# Autodesk Inventor assembly: body_8d_wid_1
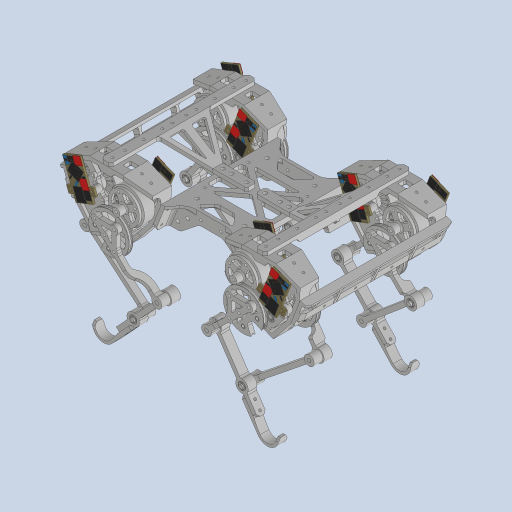
[picture p0: Inventor's stored thumbnail of the model, 512x512]
Saved by Autodesk Inventor 2023 (Build 270158000, 158)
## iProperties
Created: 2021-03-13
Part Number: body_8d_wid_1
Document SubType Name: Assembly
Designer: Shuang Peng
Author: Shuang Peng
## Documents named in this file (6)
- D:\projects-3\biped_tiny\hardware\body_8d_wid_1.iam
- D:\projects-3\biped_tiny\hardware\leg_2d_1.iam
- D:\projects-3\biped_tiny\hardware\leg_1_2d_MIR.iam
- D:\projects-3\biped_tiny\hardware\body_linker_1_wid_8d.ipt
- D:\projects-3\biped_tiny\hardware\body_linker_2_8d_wid.ipt
- D:\projects-3\biped_tiny\hardware\ex_shell_2_wid.ipt
## Components (9 placed, 5 different names)
1. leg_2d_1:1 [sub-assembly] — Insert:7, Insert:8, Flush:2
2. leg_1_2d_MIR:1 [sub-assembly] — Insert:5, Insert:6
3. leg_2d_1:2 [sub-assembly] — Insert:3, Insert:4, Insert:13, Insert:14
4. leg_1_2d_MIR:2 [sub-assembly] — Insert:1, Insert:2, Insert:15, Insert:16
5. body_linker_1_wid_8d:1 — Flush:1, Mate:1, Insert:1, Insert:2, Insert:3, Insert:4, Insert:5, Insert:6, Insert:7, Insert:8, Insert:9, Insert:10, Insert:11, Insert:12
6. body_linker_2_8d_wid:1 — Insert:9, Insert:10
7. ex_shell_2_wid:1 — Flush:2
8. body_linker_2_8d_wid:2 — Insert:11, Insert:12
9. ex_shell_2_wid:2 — Insert:13, Insert:14, Insert:15, Insert:16
## Relationships (19: Insert 16, Flush 2, Mate 1)
- Flush:1: body_linker_1_wid_8d:1
- Mate:1: body_linker_1_wid_8d:1
- Insert:1: leg_1_2d_MIR:2 ↔ body_linker_1_wid_8d:1
- Insert:2: leg_1_2d_MIR:2 ↔ body_linker_1_wid_8d:1
- Insert:3: leg_2d_1:2 ↔ body_linker_1_wid_8d:1
- Insert:4: leg_2d_1:2 ↔ body_linker_1_wid_8d:1
- Insert:5: leg_1_2d_MIR:1 ↔ body_linker_1_wid_8d:1
- Insert:6: leg_1_2d_MIR:1 ↔ body_linker_1_wid_8d:1
- Insert:7: leg_2d_1:1 ↔ body_linker_1_wid_8d:1
- Insert:8: leg_2d_1:1 ↔ body_linker_1_wid_8d:1
- Insert:9: body_linker_1_wid_8d:1 ↔ body_linker_2_8d_wid:1
- Insert:10: body_linker_1_wid_8d:1 ↔ body_linker_2_8d_wid:1
- Flush:2: leg_2d_1:1 ↔ ex_shell_2_wid:1
- Insert:11: body_linker_1_wid_8d:1 ↔ body_linker_2_8d_wid:2
- Insert:12: body_linker_1_wid_8d:1 ↔ body_linker_2_8d_wid:2
- Insert:13: leg_2d_1:2 ↔ ex_shell_2_wid:2
- Insert:14: leg_2d_1:2 ↔ ex_shell_2_wid:2
- Insert:15: leg_1_2d_MIR:2 ↔ ex_shell_2_wid:2
- Insert:16: leg_1_2d_MIR:2 ↔ ex_shell_2_wid:2
